# Autodesk Inventor assembly: shoulder_link
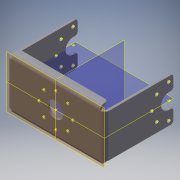
[picture p0: Inventor's stored thumbnail of the model, 180x180]
Saved by Autodesk Inventor 2018 (Build 220112000, 112)
## iProperties
Created: 2018-12-01
Part Number: shoulder_link
Document SubType Name: Assembly
Designer: jaspe
Author: jaspe
## Documents named in this file (2)
- C:\Users\jaspe\bitbots_hardware\wolfgang\assembly\arms\shoulder_link.iam
- C:\Users\jaspe\bitbots_hardware\wolfgang\assembly\body\shoulder_connector.ipt
## Components (1 placed, 1 different names)
1. shoulder_connector:1 — Mate:1, Mate:2, Angle:1
## Relationships (3: Mate 2, Angle 1)
- Mate:1: shoulder_connector:1
- Mate:2: shoulder_connector:1
- Angle:1 (90 deg): shoulder_connector:1
